# Autodesk Inventor assembly: Assembly2
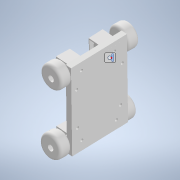
[picture p0: Inventor's stored thumbnail of the model, 180x180]
Saved by Autodesk Inventor 2020 (Build 240168000, 168)
## iProperties
Created: 2020-02-15
Part Number: Assembly2
Document SubType Name: Assembly
Designer: Hp
Author: Hp
## Documents named in this file (5)
- C:\Users\Hp\Documents\Assembly2.iam
- C:\Users\Hp\Documents\Part1.ipt
- C:\Users\Hp\Documents\s1 clamp.ipt
- C:\Users\Hp\Documents\motor.ipt
- C:\Users\Hp\Documents\wheel.ipt
## Components (13 placed, 4 different names)
1. Part1:1 — Rotational:1, Rotational:2, Rotational:3, Rotational:4
2. s1 clamp:2 — Rotational:4
3. s1 clamp:3 — Rotational:2
4. s1 clamp:4 — Rotational:1
5. s1 clamp:5 — Rotational:3, Tangent:1
6. motor:1 — Rotational:5
7. motor:2 — Tangent:1, Rotational:7
8. motor:3 — Rotational:6
9. motor:4 — Rotational:8
10. wheel:1 — Rotational:5
11. wheel:2 — Rotational:6
12. wheel:3 — Rotational:8
13. wheel:4 — Rotational:7
## Relationships (9: RevoluteJoint 8, Tangent 1)
- Rotational:1 [RevoluteJoint]: Part1:1 ↔ s1 clamp:4
- Rotational:2 [RevoluteJoint]: Part1:1 ↔ s1 clamp:3
- Rotational:3 [RevoluteJoint]: Part1:1 ↔ s1 clamp:5
- Rotational:4 [RevoluteJoint]: Part1:1 ↔ s1 clamp:2
- Tangent:1: s1 clamp:5 ↔ motor:2
- Rotational:5 [RevoluteJoint]: motor:1 ↔ wheel:1
- Rotational:6 [RevoluteJoint]: motor:3 ↔ wheel:2
- Rotational:7 [RevoluteJoint]: motor:2 ↔ wheel:4
- Rotational:8 [RevoluteJoint]: motor:4 ↔ wheel:3
